# Autodesk Inventor assembly: Assem
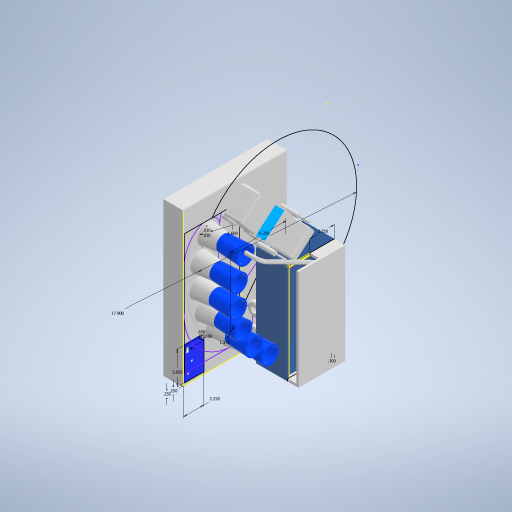
[picture p0: Inventor's stored thumbnail of the model, 512x512]
Saved by Autodesk Inventor 2024 (Build 280153000, 153)
## iProperties
Created: 2024-01-02
Part Number: Assem
Document SubType Name: Assembly
Designer: Brian
Mass: 5591.02 g
Surface Area: 11205.6 cm^2
Volume: 5587.68 cm^3
Density: 1.0006 g/cm^3
Author: Brian
## Documents named in this file (14)
- C:\Users\brian\OneDrive\Documents\Inventor\drinkSilo\Assem.iam
- C:\Users\brian\OneDrive\Documents\Inventor\drinkSilo\Micro Servo 9g.ipt
- C:\Users\brian\OneDrive\Documents\Inventor\drinkSilo\truck2.ipt
- C:\Users\brian\OneDrive\Documents\Inventor\drinkSilo\Part2.ipt
- C:\Users\brian\OneDrive\Documents\Inventor\drinkSilo\tube.ipt
- C:\Users\brian\OneDrive\Documents\Inventor\drinkSilo\truckBack.ipt
- C:\Users\brian\OneDrive\Documents\Inventor\drinkSilo\TrailerWheels.ipt
- C:\Users\brian\OneDrive\Documents\Inventor\drinkSilo\Plate.ipt
- C:\Users\brian\OneDrive\Documents\Inventor\drinkSilo\glass.ipt
- C:\Users\brian\OneDrive\Documents\Inventor\drinkSilo\lid.ipt
- C:\Users\brian\OneDrive\Documents\Inventor\drinkSilo\truckFront.ipt
- C:\Users\brian\OneDrive\Documents\Inventor\drinkSilo\Bottom.ipt
- C:\Users\brian\OneDrive\Documents\Inventor\drinkSilo\control plate.ipt
- C:\Users\brian\OneDrive\Documents\Inventor\drinkSilo\cupholder.ipt
## Components (18 placed, 13 different names)
1. Micro Servo 9g:2 — Mate:2, Rotational:2, Flush:2, Flush:3
2. truck2:1 — Rotational:1, Flush:1, Mate:1, Mate:2, Flush:2, Flush:3, Mate:5, Flush:7, Flush:8, Flush:11, Flush:12
3. Part2:1 — Rotational:2, Mate:4, Rigid:4
4. tube:1 — Mate:3, Rigid:4
5. truckBack:1 — Rotational:1, Flush:9, Mate:6, Flush:10
6. TrailerWheels:1 — Flush:1, Mate:1, Mate:10
7. Plate:1 — Mate:7, Mate:8, Mate:9, Mate:10, Mate:12, Mate:13, Insert:1, Insert:2, Mate:14, Mate:15, Mate:16
8. lid:1 — Mate:5, Flush:7, Flush:8
9. truckFront:1 — Flush:9, Mate:6, Flush:10
10. Bottom:1 — Mate:7, Mate:8, Mate:9, Flush:11, Flush:12, Mate:12, Mate:13
11. control plate:1 — Mate:14, Mate:15, Mate:16
12. cupholder:1 — Insert:1, Insert:2
13. glass:1
14. glass:2
15. glass:3
16. glass:4
17. glass:5
18. glass:6
## Component patterns: (6 elements, first: glass:1)
## Relationships (29: Mate 15, Flush 9, RevoluteJoint 2, Insert 2, WeldJoint 1)
- Rotational:1 [RevoluteJoint] (6.35 mm): truck2:1 ↔ truckBack:1
- Flush:1: truck2:1 ↔ TrailerWheels:1
- Mate:1: truck2:1 ↔ TrailerWheels:1
- Mate:2: Micro Servo 9g:2 ↔ truck2:1
- Rotational:2 [RevoluteJoint]: Micro Servo 9g:2 ↔ Part2:1
- Flush:2: Micro Servo 9g:2 ↔ truck2:1
- Flush:3: Micro Servo 9g:2 ↔ truck2:1
- Mate:3: tube:1
- Mate:4: Part2:1
- Mate:5: truck2:1 ↔ lid:1
- Flush:7: truck2:1 ↔ lid:1
- Flush:8: truck2:1 ↔ lid:1
- Flush:9: truckBack:1 ↔ truckFront:1
- Mate:6: truckBack:1 ↔ truckFront:1
- Flush:10 (-14.605 mm): truckBack:1 ↔ truckFront:1
- Mate:7: Plate:1 ↔ Bottom:1
- Mate:8: Plate:1 ↔ Bottom:1
- Mate:9: Plate:1 ↔ Bottom:1
- Rigid:4 [WeldJoint] (3.81 mm): Part2:1 ↔ tube:1
- Flush:11: truck2:1 ↔ Bottom:1
- Mate:10 (19.05 mm): TrailerWheels:1 ↔ Plate:1
- Flush:12: truck2:1 ↔ Bottom:1
- Mate:12: Plate:1 ↔ Bottom:1
- Mate:13: Plate:1 ↔ Bottom:1
- Insert:1 (1.27 mm): Plate:1 ↔ cupholder:1
- Insert:2 (1.27 mm): Plate:1 ↔ cupholder:1
- Mate:14 (-1 mm): Plate:1 ↔ control plate:1
- Mate:15 (1.27 mm): Plate:1 ↔ control plate:1
- Mate:16 (1.27 mm): Plate:1 ↔ control plate:1
